# Autodesk Inventor assembly: Assembly2
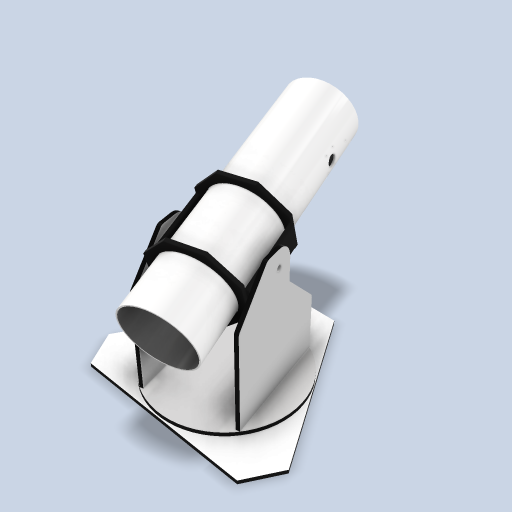
[picture p0: Inventor's stored thumbnail of the model, 512x512]
Saved by Autodesk Inventor 2023 (Build 270158000, 158)
## iProperties
Created: 2022-10-16
Part Number: Assembly2
Document SubType Name: Assembly
Designer: Nathan
Author: Nathan
## Documents named in this file (8)
- C:\Users\Nathan\Desktop\Senior Project\Schematics\Parts\Assembly2.iam
- C:\Users\Nathan\Desktop\Senior Project\Schematics\Parts\Triangle Base.ipt
- C:\Users\Nathan\Desktop\Senior Project\Schematics\Parts\base turntable.ipt
- C:\Users\Nathan\Desktop\Senior Project\Schematics\Parts\base side.ipt
- C:\Users\Nathan\Desktop\Senior Project\Schematics\Parts\12in lazy susan.iam
- C:\Users\Nathan\Desktop\Senior Project\Schematics\Parts\Tube Ring Joiner.ipt
- C:\Users\Nathan\Desktop\Senior Project\Schematics\Parts\Bracket.ipt
- C:\Users\Nathan\Desktop\Senior Project\Schematics\Parts\tube.ipt
## Components (10 placed, 7 different names)
1. Triangle Base:1 — Mate:6, Mate:7, Tangent:1, Tangent:2
2. base turntable:1 — Mate:1, Mate:2, Mate:3, Mate:4, Mate:5, Mate:8, Tangent:1, Tangent:2, Angle:1
3. base side:1 — Mate:4, Mate:5, Angle:1, Rotational:1
4. base side:2 — Mate:1, Mate:2, Mate:3, Rotational:2, Angle:3
5. 12in lazy susan:1 [sub-assembly] — Mate:6, Mate:7, Mate:8
6. Tube Ring Joiner:1 — Mate:11, Flush:1, Rotational:1, Mate:12, Mate:14, Mate:16
7. Tube Ring Joiner:2 — Rotational:2, Mate:13, Mate:15, Mate:17
8. Bracket:1 — Mate:14, Mate:15, Mate:16, Mate:17, Insert:1, Angle:2
9. Bracket:2 — Mate:11, Flush:1, Mate:12, Mate:13
10. tube:1 — Insert:1, Angle:2, Angle:3
## Relationships (24: Mate 15, Angle 3, Tangent 2, RevoluteJoint 2, Flush 1, Insert 1)
- Mate:1: base turntable:1 ↔ base side:2
- Mate:2: base turntable:1 ↔ base side:2
- Mate:3: base turntable:1 ↔ base side:2
- Mate:4: base turntable:1 ↔ base side:1
- Mate:5: base turntable:1 ↔ base side:1
- Mate:6: Triangle Base:1 ↔ 12in lazy susan:1
- Mate:7: Triangle Base:1 ↔ 12in lazy susan:1
- Mate:8: base turntable:1 ↔ 12in lazy susan:1
- Tangent:1: Triangle Base:1 ↔ base turntable:1
- Tangent:2: Triangle Base:1 ↔ base turntable:1
- Angle:1 (-90 deg): base turntable:1 ↔ base side:1
- Mate:11: Tube Ring Joiner:1 ↔ Bracket:2
- Flush:1: Tube Ring Joiner:1 ↔ Bracket:2
- Rotational:1 [RevoluteJoint] (-36.0172 mm): base side:1 ↔ Tube Ring Joiner:1
- Mate:12 (29.21 mm): Tube Ring Joiner:1 ↔ Bracket:2
- Rotational:2 [RevoluteJoint] (-18.0086 mm): base side:2 ↔ Tube Ring Joiner:2
- Mate:13: Tube Ring Joiner:2 ↔ Bracket:2
- Mate:14: Tube Ring Joiner:1 ↔ Bracket:1
- Mate:15: Tube Ring Joiner:2 ↔ Bracket:1
- Mate:16: Tube Ring Joiner:1 ↔ Bracket:1
- Mate:17 (29.21 mm): Tube Ring Joiner:2 ↔ Bracket:1
- Insert:1 (889 mm): Bracket:1 ↔ tube:1
- Angle:2 (270 deg): Bracket:1 ↔ tube:1
- Angle:3 (0 deg): base side:2 ↔ tube:1
